# Autodesk Inventor assembly: Piston
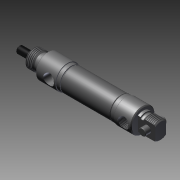
[picture p0: Inventor's stored thumbnail of the model, 180x180]
Saved by Autodesk Inventor 2015 (Build 190159000, 159)
## iProperties
Category: PARTsolutions
Company: BIMBA
Created: 2015-01-23
Part Number: Piston
Catalog Web Link: www.cadenas.de
Description: Original Line Standard Air Cylinders-
Vendor: BIMBA
Document SubType Name: Assembly
Designer: psAdmin
Manufacturer: BIMBA
PSOL_IDENT_0: {$CADENAS_DATA\23d-libs\bimba\bimba\bimba_imperial\bimba_full_line\original_line_cylinders\standard_
PSOL_IDENT_1: air_cylinders\standard_air_cylinder_asmtab.prj},323 {VTYP=3D},{STYP=ASSTAB},{NB=040.5-DP(F,D-9)},{LI
PSOL_IDENT_2: NA=040.5-DP},{NN=Original Line Standard Air Cylinders},{DATE=08.09.2014 04:47:41},{GEOMDATE=08.09.20
PSOL_IDENT_3: 14 04:47:39},{VERSION=},{LINEID=50},{LINESUBID=-1},{WBVAR=STROKE,ACTING,MNT,DER,NR,BM,CO,OO,VO,M,EE,
PSOL_IDENT_4: EEL,K,Q,Y,G,T,B,H,SER,SR,NT,W,HL,STPT1,STPT2,STPT3,STPT4,MB,PB,PRC,TB,MN}  {NB=040.5-DP(F,D-9)},{LIN
PSOL_IDENT_5: A=040.5-DP},{KT=DUMMY},{PN=040.5-DP},{PNC=040.5-DP(F,D-9)},{PNA=(D-9)},{DASH=-},{BORE1=0.75000000},{
PSOL_IDENT_6: BORE=3/4\" (04)},{BOREPN=04},{STROKE=0.500},{STROKEALG=[0.011:50/0.001]},{STROKE1=0.500},{ACTING=D},
PSOL_IDENT_7: {ACTINGALG= '' , 'Single Acting (SA)' , 'R' , 'Reverse Single Acting (SA)' , 'D' , 'Double Acting (S
PSOL_IDENT_8: A)' },{ACTINGPN=D},{MNT=P},{MNTALG= '' , 'Front Nose Mounting (SA)' , 'P' , 'Rear Pivot Mounting (SA
PSOL_IDENT_9: )' , 'XP' , 'Double End or Pivot Mounting (SA)' , 'X' , 'Double End Mounting (SA)' , 'BF' , 'Front B
PSOL_IDENT_10: lock Mounting (SA)' , 'BR' , 'Rear Block Mounting for Vertical Positioning (SA)' , 'BFT' , 'Front Bl
PSOL_IDENT_11: ock Trunnion Mounting (SA)' , 'BRT' , 'Rear Block Trunnion Mounting (SA)' },{TYPE=},{MNTPN=P},{DER=}
PSOL_IDENT_12: ,{DERALG= '' , 'N/A' },{NR=},{NRALG= '' , 'N/A' },{NRPN=},{BM=},{BMALG= '' , 'N/A' },{BMPN=},{CO=},{
PSOL_IDENT_13: COALG= '' , 'N/A' },{OO=},{OOALG= '', 'N/A' },{OOPN=},{VO=Z},{VOALG= 'Z' , 'N/A' },{VOPN=},{OOVOPN=}
PSOL_IDENT_14: ,{M=},{MALG= '', 'Without Magnet', 'M', 'With Magnet' },{EE=},{EEL=0.000},{EEMAX=49.5000},{EEALG= ''
PSOL_IDENT_15: , 'Without Extra Extension', 'EE', 'With Extra Extension' },{EELALG=0},{EEPN=},{EEPN1=0.000},{K=},{K
PSOL_IDENT_16: ALG= '', 'Standard' , 'K' , 'Ports Rotated 90deg K' },{KPN=},{Q=},{QALG= '' , 'N/A' },{QPN=},{Y=},{Y
PSOL_IDENT_17: ALG= '' , 'Without Pivot Bushing' , 'Y' , 'With Pivot Bushing' },{YPN=},{YCON=},{F=},{FALG= '', 'Non
PSOL_IDENT_18: -Coated (Standard)', 'F', 'Molycoated' },{FPN=},{G=},{GPN=},{GPN99=},{T=},{TALG= '' , 'Standard -20°
PSOL_IDENT_19: to 200°F (-29° to 95°C)' , 'N' , 'Low Temperature' , 'V' , 'High Temperature' },{NPN=},{VPN=},{B=},
PSOL_IDENT_20: {BALG= '', 'W/out Bumpers' , 'B' , 'W/ Bumpers' },{BPN=},{H=},{HALG= '', 'N/A' },{HPN=},{SER=},{SERA
PSOL_IDENT_21: LG= '' , 'Without Spring Extend/Return' , 'JS' , 'With Spring Return' , 'JR' , 'With Spring Extend'
PSOL_IDENT_22: },{SR=C},{SRALG= 'C' , 'Standard Blackened Carbon Steel' , 'SR' , 'Stainless Steel [SR]' },{SRPN=},{
PSOL_IDENT_23: SRCON=1},{NT=},{NTPN=},{W=},{WALG= '' , 'Without Wiper' , 'W' , 'With Wiper' },{WPN=},{E=},{EALG= ''
PSOL_IDENT_24: , 'Standard Seals/Lube' , 'E' , 'Non-Lube Seals/Lube' },{EPN=},{HL=},{HLALG= '' , 'Without Low Pres
PSOL_IDENT_25: sure Hydraulic' , 'HL' , 'With Low Pressure Hydraulic' },{ST=},{STALG= '' , 'N/A' },{STPT1=},{STPT1A
PSOL_IDENT_26: LG= '' , 'N/A' },{STPT2=},{STPT2ALG= '' , 'N/A' },{STPT3=},{STPT3ALG= '' , 'N/A' },{STPT4=},{STPT4AL
PSOL_IDENT_27: G= '' , 'N/A' },{STPN=},{MB=},{MBALG= '' , 'N/A' },{MBPN=},{MBPNALL=},{MBPNALLREAR=},{PB=},{PBALG= ''
PSOL_IDENT_28: , 'Without Pivot Bracket' , 'D-167' , 'D-167' },{PBPN=},{PBPNALL=D-167},{PRC=},{PRCALG= '' , 'W/out
PSOL_IDENT_29: Pivot Rod Clevis' , 'F,D-166-3' , 'D-166-3 (front)' },{PRCPN=},{PRCPNALL=D-166-3},{TB=},{TBALG= ''
PSOL_IDENT_30: , 'N/A' },{TBPN=},{TBPNALL=},{MN=F,D-9},{MNALG= '' , 'Without Mounting Nut' , 'F,D-9' , 'D-9 (front)'
PSOL_IDENT_31: , 'R,D-9' , 'D-9 (rear)', '2x,D-9' , 'D-9 (front & rear)' },{MNPN=(F,D-9)},{MNCONF=D-9},{MNCONR=},{
PSOL_IDENT_32: TLEN=1.7555},{FRAC=3.7500},{RGCON=},{RGDACCON=R},{RHCON=P},{RHCON1=P},{RHCONON=1},{RHACCON=},{FNUTCO
PSOL_IDENT_33: N=1},{RNUTCON=0},{FNUTPN=D-9},{RNUTPN=D-9},{FNUTTRANS=0.0000},{RNUTTRANS=0.0000},{VHOLECON=0},{A1=1.
PSOL_IDENT_34: 5940},{A1N=0.8750},{A1P=1.5940},{A1B=1.5940},{A4=0.2525},{A4N=0.3130},{A4P=0.2525},{A5=0.0300},{A1H=
PSOL_IDENT_35: 1.594},{A1NH=0.5310},{A1PH=1.5940},{A1BH=1.0940},{A1SH=1.2190},{A2H=0.2190},{A2NH=0.2190},{LENGTH=3.
PSOL_IDENT_36: 7500},{LENGTH1=3.7500},{LENGTH2=3.8100},{MUL=0.5000},{MUL11=0.5000},{MUL22=1.345},{MUL33=0.8450},{MU
PSOL_IDENT_37: L2=0.5000},{MUL211=0.5000},{MUL222=2.6900},{MUL233=1.6900},{SSS=0.5000},{RGLEN=1.3715},{RHLEN=1.1230
PSOL_IDENT_38: },{SSS1=1.0000},{A13=1.3120},{DIF=0.0000},{G5=0.6250},{ON=0},{SSADD=0.0000},{BADD=0.0000},{MADD=0.00
PSOL_IDENT_39: 00},{NVADD=0.0000},{TRACKL=1.4655},{TRACKCON=D-74168},{TRIMCON=0},{TRIMCON1=0},{PINCON=D-51},{FSPACE=
PSOL_IDENT_40: 0.6604},{SPACE=0.0482},{TEXT=0.0844},{S1=1.0000},{D1=0.8325},{D1N=0.8050},{D1B=0.8625},{D1P=0.8325},
PSOL_IDENT_41: {FA=0.940},{RA=0.9400},{PPATH=standard_air_cylinder_asmtpl.prj},{MATALGHTML=<b>Standard Original Lin
PSOL_IDENT_42: e:</b><dl><dt>Rod:</dt><dd>- Stainless Steel</dd><dd>&nbsp;&nbsp;(5/16 9/16 Bores)</dd><dd>- High St
PSOL_IDENT_43: rength Carbon Steel</dd><dd>&nbsp;&nbsp;(3/4 3 Bore)</dd><dd>- Stainless Steel</dd><dd>&nbsp;&nbsp;(
PSOL_IDENT_44: X style DXP/DX/DXDE)</dd><dt>Bearings:</dt><dd>- Sintered Bronze</dd><dt>Body:</dt><dd>- 304 Stainle
PSOL_IDENT_45: ss Steel</dd><dt>End Caps:</dt><dd>- Aluminum</dd><dt>Seals:</dt><dd>- Buna N</dd></dl>},{ASSCFGPRA=
PSOL_IDENT_46: 04DP},{MBPNA=},{MNPNA=(D-9)},{PRCPNA=},{ASSOPTACC=STPT4},{A=4.25},{HADD=0.0000},{WFL=0.25},{QADD=0.0
PSOL_IDENT_47: 00},{QADD1=0.440},{TEST=0.0000},{MNTB=},{STDNUTF=0},{STDNUTR=0}
SUPPLIER: BIMBA
ARTICLENO: 040.5-DP(F,D-9)
BOMINFO: 040.5-DP
CREATOR: CADENAS GmbH
Title: 040.5-DP
Author: Cadenas PARTsolutions
## Documents named in this file (7)
- C:\Users\Brian\Documents\Inventor\FRC\Extender\040  .5d\Piston.iam
- C:\Users\Brian\Documents\Inventor\FRC\Extender\040  .5d\040_5_DPC_F_D_9_0000_0_dummy.ipt
- C:\Users\Brian\Documents\Inventor\FRC\Extender\040  .5d\04R000_0_rod_guide.ipt
- C:\Users\Brian\Documents\Inventor\FRC\Extender\040  .5d\04R_1_75550C.ipt
- C:\Users\Brian\Documents\Inventor\FRC\Extender\040  .5d\04P0000_rear_head.ipt
- C:\Users\Brian\Documents\Inventor\FRC\Extender\040  .5d\D_51.ipt
- C:\Users\Brian\Documents\Inventor\FRC\Extender\040  .5d\C_040_5_DP0_rod.ipt
## Components (6 placed, 6 different names)
1. 040_5_DPC_F_D_9_0000_0_dummy:1
2. 04R000_0_rod_guide:1 — Mate:1
3. 04R_1_75550C:1
4. 04P0000_rear_head:1
5. D_51:1
6. C_040_5_DP0_rod:1 — Mate:1
## Relationships (1: Mate 1)
- Mate:1: 04R000_0_rod_guide:1 ↔ C_040_5_DP0_rod:1
